# Autodesk Inventor assembly: slide
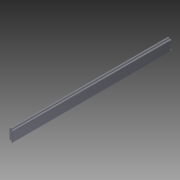
[picture p0: Inventor's stored thumbnail of the model, 180x180]
Saved by Autodesk Inventor 2012 (Build 160160000, 160)
## iProperties
Created: 2011-12-02
Part Number: slide
Document SubType Name: Assembly
Designer: Antonella
Author: Antonella
## Documents named in this file (3)
- C:\Users\Antonella\Documents\GCC Robotics 2012 - Mechanical\Robot 2.0\Payload Mount\slide.iam
- C:\Users\Antonella\Documents\GCC Robotics 2012 - Mechanical\Robot 2.0\Payload Mount\slide inner.ipt
- C:\Users\Antonella\Documents\GCC Robotics 2012 - Mechanical\Robot 2.0\Payload Mount\slide outer.ipt
## Components (2 placed, 2 different names)
1. slide outer:1 — Mate:1, Mate:2
2. slide inner:1 — Mate:1, Mate:2
## Relationships (2: Mate 2)
- Mate:1: slide outer:1 ↔ slide inner:1
- Mate:2: slide outer:1 ↔ slide inner:1
